# Autodesk Inventor assembly: B_Drive
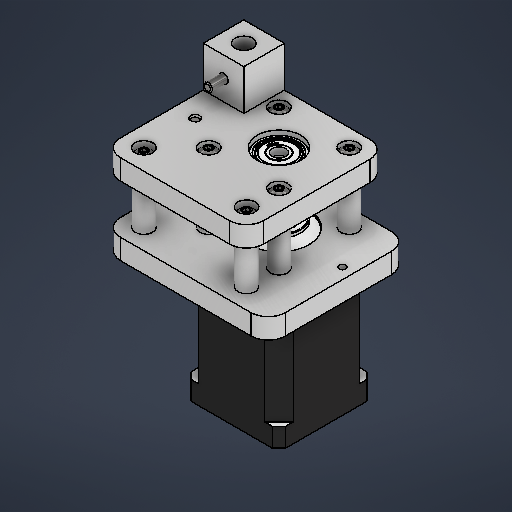
[picture p0: Inventor's stored thumbnail of the model, 512x512]
Saved by Autodesk Inventor 2026 (Build 300175050, 175E)
## iProperties
Created: 2025-05-24
Part Number: B_Drive
Document SubType Name: Assembly
Designer: Joshua Eah
Author: Joshua Eah
## Documents named in this file (14)
- C:\Users\Joshua Eah\Documents\GitHub\Voron-0\CAD\Tulip - Machined Parts\AB Drives\B Drive\B_Drive.iam
- C:\Users\Joshua Eah\Documents\GitHub\Voron-0\CAD\Tulip - Machined Parts\AB Drives\B Drive\B Drive Frame Lower (Tulip).ipt
- C:\Users\Joshua Eah\Documents\GitHub\Voron-0\CAD\Machined Parts\Spacers\Spacer.ipt
- C:\Users\Joshua Eah\Documents\GitHub\Voron-0\CAD\Tulip - Machined Parts\AB Drives\Drive Frame Spacer\Drive Frame Spacer.ipt
- C:\Users\Joshua Eah\Documents\GitHub\Voron-0\CAD\Tulip - Machined Parts\AB Drives\B Drive\B Drive Frame Upper (Tulip).ipt
- C:\Users\Joshua Eah\Documents\GitHub\Voron-0\CAD\Master Assembly\Hardware\3x30 Pin.ipt
- C:\Users\Joshua Eah\Documents\GitHub\Voron-0\CAD\Master Assembly\Hardware\F623 Stack.iam
- C:\Users\Joshua Eah\Documents\GitHub\Voron-0\CAD\Master Assembly\Hardware\M3x35 BHCS.ipt
- C:\Users\Joshua Eah\Documents\GitHub\Voron-0\CAD\Master Assembly\Hardware\M3x30 BHCS.ipt
- C:\Users\Joshua Eah\Documents\GitHub\Voron-0\CAD\Master Assembly\Hardware\M3_Washer.ipt
- C:\Users\Joshua Eah\Documents\GitHub\Voron-0\CAD\Master Assembly\Hardware\M3x10 BHCS.ipt
- C:\Users\Joshua Eah\Documents\GitHub\Voron-0\CAD\Master Assembly\AB Drives\Motor Assembly\Nema14.ipt
- C:\Users\Joshua Eah\Documents\GitHub\Voron-0\CAD\Tulip - Machined Parts\V0.2R1 Tulip Mod master v35\625 - ZZ Bearing v1 (2).iam
- C:\Users\Joshua Eah\Documents\GitHub\Voron-0\CAD\Master Assembly\AB Drives\Motor Assembly\GT2 20T 6mm Pulley.iam
## Components (29 placed, 13 different names)
1. B Drive Frame Lower (Tulip):1 — Insert:1, Insert:2, Insert:3, Insert:4, Insert:5, Insert:6, Insert:7, Insert:10, Insert:11, Insert:14, Insert:25, Insert:27, Insert:28
2. Spacer:1 — Insert:1, Insert:12
3. Drive Frame Spacer:1 — Insert:2
4. Drive Frame Spacer:2 — Insert:3
5. Drive Frame Spacer:3 — Insert:4
6. Drive Frame Spacer:4 — Insert:5, Insert:9
7. Drive Frame Spacer:5 — Insert:6
8. Drive Frame Spacer:6 — Insert:7, Insert:8
9. B Drive Frame Upper (Tulip):1 — Insert:8, Insert:9, Mate:1, Mate:2, Insert:15, Insert:16, Insert:21, Insert:22, Insert:23, Insert:24, Insert:26, Insert:29
10. 3x30 Pin:1 — Mate:1, Insert:10
11. 3x30 Pin:2 — Mate:2, Insert:11
12. F623 Stack:1 [sub-assembly] — Insert:12
13. F623 Stack:2 [sub-assembly] — Insert:13, Insert:14
14. F623 Stack:3 [sub-assembly] — Insert:13
15. M3x35 BHCS:1 — Insert:15
16. M3x35 BHCS:2 — Insert:16
17. M3x30 BHCS:1 — Insert:17
18. M3_Washer:1 — Insert:17, Insert:21
19. M3x30 BHCS:2
20. M3_Washer:2 — Insert:22
21. M3x30 BHCS:3
22. M3_Washer:3 — Insert:23
23. M3x30 BHCS:4
24. M3_Washer:4 — Insert:24
25. M3x10 BHCS:1 — Insert:25
26. M3x10 BHCS:2 — Insert:26
27. Nema14:1 — Insert:27, Insert:28, Mate:3, Mate:4
28. 625 - ZZ Bearing v1 (2):1 [sub-assembly] — Insert:29
29. GT2 20T 6mm Pulley:1 [sub-assembly] — Mate:3, Mate:4
## Relationships (33: Insert 29, Mate 4)
- Insert:1: B Drive Frame Lower (Tulip):1 ↔ Spacer:1
- Insert:2: B Drive Frame Lower (Tulip):1 ↔ Drive Frame Spacer:1
- Insert:3: B Drive Frame Lower (Tulip):1 ↔ Drive Frame Spacer:2
- Insert:4: B Drive Frame Lower (Tulip):1 ↔ Drive Frame Spacer:3
- Insert:5: B Drive Frame Lower (Tulip):1 ↔ Drive Frame Spacer:4
- Insert:6: B Drive Frame Lower (Tulip):1 ↔ Drive Frame Spacer:5
- Insert:7: B Drive Frame Lower (Tulip):1 ↔ Drive Frame Spacer:6
- Insert:8: Drive Frame Spacer:6 ↔ B Drive Frame Upper (Tulip):1
- Insert:9: Drive Frame Spacer:4 ↔ B Drive Frame Upper (Tulip):1
- Mate:1: B Drive Frame Upper (Tulip):1 ↔ 3x30 Pin:1
- Mate:2: B Drive Frame Upper (Tulip):1 ↔ 3x30 Pin:2
- Insert:10: B Drive Frame Lower (Tulip):1 ↔ 3x30 Pin:1
- Insert:11: B Drive Frame Lower (Tulip):1 ↔ 3x30 Pin:2
- Insert:12: Spacer:1 ↔ F623 Stack:1
- Insert:13: F623 Stack:2 ↔ F623 Stack:3
- Insert:14: B Drive Frame Lower (Tulip):1 ↔ F623 Stack:2
- Insert:15: B Drive Frame Upper (Tulip):1 ↔ M3x35 BHCS:1
- Insert:16: B Drive Frame Upper (Tulip):1 ↔ M3x35 BHCS:2
- Insert:17: M3x30 BHCS:1 ↔ M3_Washer:1
- [Insert]: M3x30 BHCS:2 ↔ M3_Washer:2
- [Insert]: M3x30 BHCS:3 ↔ M3_Washer:3
- [Insert]: M3x30 BHCS:4 ↔ M3_Washer:4
- Insert:21: B Drive Frame Upper (Tulip):1 ↔ M3_Washer:1
- Insert:22: B Drive Frame Upper (Tulip):1 ↔ M3_Washer:2
- Insert:23: B Drive Frame Upper (Tulip):1 ↔ M3_Washer:3
- Insert:24: B Drive Frame Upper (Tulip):1 ↔ M3_Washer:4
- Insert:25: B Drive Frame Lower (Tulip):1 ↔ M3x10 BHCS:1
- Insert:26: B Drive Frame Upper (Tulip):1 ↔ M3x10 BHCS:2
- Insert:27: B Drive Frame Lower (Tulip):1 ↔ Nema14:1
- Insert:28: B Drive Frame Lower (Tulip):1 ↔ Nema14:1
- Insert:29: B Drive Frame Upper (Tulip):1 ↔ 625 - ZZ Bearing v1 (2):1
- Mate:3: Nema14:1 ↔ GT2 20T 6mm Pulley:1
- Mate:4 (2.65 mm): Nema14:1 ↔ GT2 20T 6mm Pulley:1
## Named parameters: d19_d18 = 0 mm, d20_d18 = 0 mm, d21_d18 = 0 mm
